# Autodesk Inventor assembly: Right Front Wheel with hub
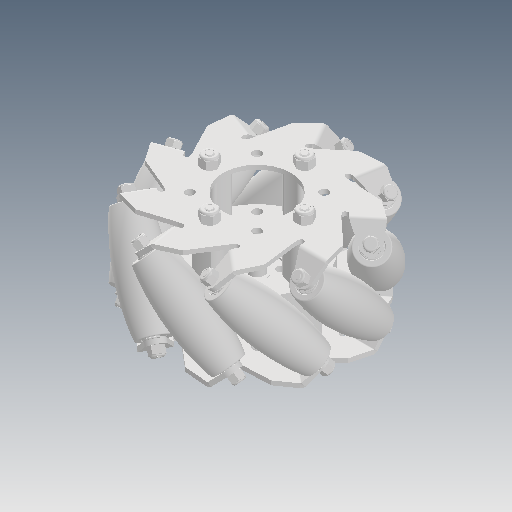
[picture p0: Inventor's stored thumbnail of the model, 512x512]
Saved by Autodesk Inventor 2020 (Build 240168000, 168)
## iProperties
Created: 2020-02-22
Part Number: Right Front Wheel with hub
Document SubType Name: Assembly
Designer: ball
Author: ball
## Documents named in this file (5)
- C:\FTC\FTC8863CAD\2019 Robot\Mecanum Drive Train Metal\Right Front Wheel with hub.iam
- C:\FTC\FTC8863CAD\GoBilda\3213 Parts\3606-0100-0100 assembly.iam
- C:\FTC\FTC8863CAD\GoBilda\1310 Parts\1310-0016-4008 assembly.ipt
- C:\FTC\FTC8863CAD\StepLibraries\Screws\M4 x 22 SOCKET HEAD CAP SCREW.ipt
- C:\FTC\FTC8863CAD\StepLibraries\Washers\M4 FLAT WASHER.ipt
## Components (10 placed, 4 different names)
1. 3606-0100-0100 assembly:1 [sub-assembly] — Mate:1, Mate:2, Mate:3, Mate:20, Mate:21, Mate:22, Mate:23, Mate:24, Mate:25, Mate:26, Mate:27
2. 1310-0016-4008 assembly:1 — Mate:1, Mate:2, Mate:3
3. M4 x 22 SOCKET HEAD CAP SCREW:5 — Mate:12, Mate:13, Mate:21
4. M4 FLAT WASHER:1 — Mate:12, Mate:13, Mate:20
5. M4 x 22 SOCKET HEAD CAP SCREW:6 — Mate:23
6. M4 FLAT WASHER:2 — Mate:22
7. M4 x 22 SOCKET HEAD CAP SCREW:7 — Mate:26
8. M4 FLAT WASHER:3 — Mate:25
9. M4 x 22 SOCKET HEAD CAP SCREW:8 — Mate:27
10. M4 FLAT WASHER:4 — Mate:24
## Relationships (19: Mate 19)
- Mate:1: 3606-0100-0100 assembly:1 ↔ 1310-0016-4008 assembly:1
- Mate:2: 3606-0100-0100 assembly:1 ↔ 1310-0016-4008 assembly:1
- Mate:3: 3606-0100-0100 assembly:1 ↔ 1310-0016-4008 assembly:1
- Mate:12: M4 x 22 SOCKET HEAD CAP SCREW:5 ↔ M4 FLAT WASHER:1
- Mate:13: M4 x 22 SOCKET HEAD CAP SCREW:5 ↔ M4 FLAT WASHER:1
- [Mate]: M4 x 22 SOCKET HEAD CAP SCREW:6 ↔ M4 FLAT WASHER:2
- [Mate]: M4 x 22 SOCKET HEAD CAP SCREW:6 ↔ M4 FLAT WASHER:2
- [Mate]: M4 x 22 SOCKET HEAD CAP SCREW:7 ↔ M4 FLAT WASHER:3
- [Mate]: M4 x 22 SOCKET HEAD CAP SCREW:7 ↔ M4 FLAT WASHER:3
- [Mate]: M4 x 22 SOCKET HEAD CAP SCREW:8 ↔ M4 FLAT WASHER:4
- [Mate]: M4 x 22 SOCKET HEAD CAP SCREW:8 ↔ M4 FLAT WASHER:4
- Mate:20: 3606-0100-0100 assembly:1 ↔ M4 FLAT WASHER:1
- Mate:21: 3606-0100-0100 assembly:1 ↔ M4 x 22 SOCKET HEAD CAP SCREW:5
- Mate:22: 3606-0100-0100 assembly:1 ↔ M4 FLAT WASHER:2
- Mate:23: 3606-0100-0100 assembly:1 ↔ M4 x 22 SOCKET HEAD CAP SCREW:6
- Mate:24: 3606-0100-0100 assembly:1 ↔ M4 FLAT WASHER:4
- Mate:25: 3606-0100-0100 assembly:1 ↔ M4 FLAT WASHER:3
- Mate:26: 3606-0100-0100 assembly:1 ↔ M4 x 22 SOCKET HEAD CAP SCREW:7
- Mate:27: 3606-0100-0100 assembly:1 ↔ M4 x 22 SOCKET HEAD CAP SCREW:8
## Named parameters: d14_d12 = 0 mm, d15_d13 = 0 mm, d16_d12 = 0 mm, d17_d13 = 0 mm, d18_d12 = 0 mm, d19_d13 = 0 mm
